# Autodesk Inventor assembly: bearings_MIR
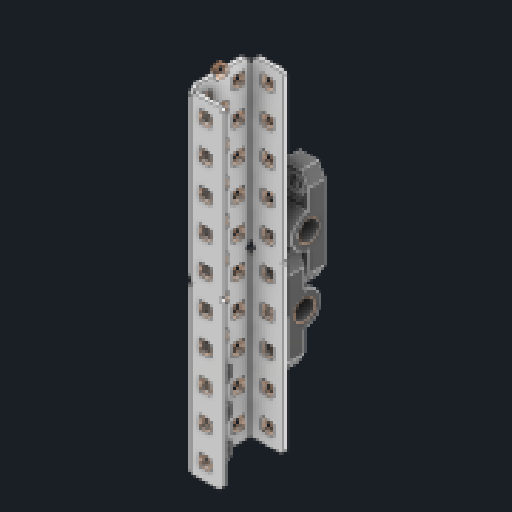
[picture p0: Inventor's stored thumbnail of the model, 512x512]
Saved by Autodesk Inventor 2024 (Build 280153000, 153)
## iProperties
Created: 2023-08-16
Part Number: bearings_MIR
Document SubType Name: Assembly
Designer: avere
Author: avere
## Documents named in this file (11)
- D:\vex_robotics\hardware\cad\scrap_v0.1\catapult\mirrored_parts\bearings_MIR.iam
- D:\vex_robotics\hardware\cad\scrap_v0.1\catapult\mirrored_parts\Alu C 1x2x1x10_MIR.ipt
- D:\vex_robotics\hardware\cad\scrap_v0.1\catapult\mirrored_parts\Bearing Flat Low Profile_MIR.ipt
- D:\vex_robotics\hardware\cad\scrap_v0.1\catapult\mirrored_parts\HS Pillow Bearing Block_MIR.ipt
- D:\vex_robotics\hardware\cad\VEX-CAD-Inventor-1.41\Structure\Hardware\Nut Nylon\Nut Nylon - White.ipt
- D:\vex_robotics\hardware\cad\VEX-CAD-Inventor-1.41\Structure\Hardware\Nut Nylon.ipt
- D:\vex_robotics\hardware\cad\VEX-CAD-Inventor-1.41\Motion\Spacers\Spacer Nylon .375 OD.ipt
- D:\vex_robotics\hardware\cad\VEX-CAD-Inventor-1.41\Motion\Spacers\Spacer Nylon .375 OD\NSpacer .375 OD x .250.ipt
- D:\vex_robotics\hardware\cad\VEX-CAD-Inventor-1.41\Motion\Spacers\Washer Steel\SWasher .375 OD x .062500.ipt
- D:\vex_robotics\hardware\cad\VEX-CAD-Inventor-1.41\Motion\Spacers\Washer Steel.ipt
- D:\vex_robotics\hardware\cad\VEX-CAD-Inventor-1.41\Motion\Spacers\Washer Steel\SWasher .375 OD x .015625.ipt
## Components (8 placed, 7 different names)
1. Alu C 1x2x1x10_MIR:1 — Mate:1, Insert:1, Insert:2, Mate:2
2. Bearing Flat Low Profile_MIR:1 — Mate:1, Insert:1
3. HS Pillow Bearing Block_MIR:1 — Insert:2, Mate:2, Mate:3, Insert:5
4. HS Pillow Bearing Block_MIR:2 — Insert:4, Mate:3, Insert:5
5. Nut Nylon - White:1 — Insert:4, Insert:6
6. NSpacer .375 OD x .250:2 — Insert:6, Insert:8
7. SWasher .375 OD x .062500:1 — Insert:7
8. SWasher .375 OD x .015625:2 — Insert:7, Insert:8
## Relationships (10: Insert 7, Mate 3)
- Mate:1: Alu C 1x2x1x10_MIR:1 ↔ Bearing Flat Low Profile_MIR:1
- Insert:1: Alu C 1x2x1x10_MIR:1 ↔ Bearing Flat Low Profile_MIR:1
- Insert:2: Alu C 1x2x1x10_MIR:1 ↔ HS Pillow Bearing Block_MIR:1
- Mate:2: Alu C 1x2x1x10_MIR:1 ↔ HS Pillow Bearing Block_MIR:1
- Insert:4: HS Pillow Bearing Block_MIR:2 ↔ Nut Nylon - White:1
- Mate:3: HS Pillow Bearing Block_MIR:1 ↔ HS Pillow Bearing Block_MIR:2
- Insert:5 (9.525 mm): HS Pillow Bearing Block_MIR:1 ↔ HS Pillow Bearing Block_MIR:2
- Insert:6: Nut Nylon - White:1 ↔ NSpacer .375 OD x .250:2
- Insert:7: SWasher .375 OD x .062500:1 ↔ SWasher .375 OD x .015625:2
- Insert:8: NSpacer .375 OD x .250:2 ↔ SWasher .375 OD x .015625:2
